# Autodesk Inventor assembly: sestava estonsko
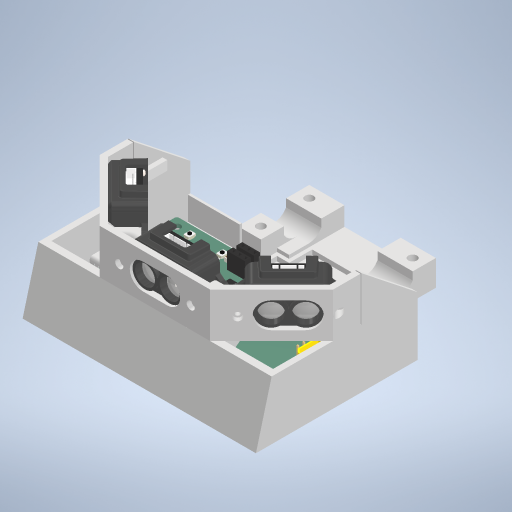
[picture p0: Inventor's stored thumbnail of the model, 512x512]
Saved by Autodesk Inventor 2024 (Build 280153000, 153)
## iProperties
Created: 2023-10-31
Part Number: sestava estonsko
Document SubType Name: Assembly
Designer: Simak
Author: Simak
## Documents named in this file (4)
- C:\Users\jaryj\Desktop\Škola\Mini sumo\RoboCop\- 3D -\wip\sestava estonsko.iam
- C:\Users\jaryj\Desktop\Škola\Mini sumo\RoboCop\- 3D -\el._parts\sumec\sumec.ipt
- C:\Users\jaryj\Desktop\Škola\Mini sumo\RoboCop\- 3D -\wip\tělo estonsko.ipt
- C:\Users\jaryj\Desktop\Škola\Mini sumo\RoboCop\- 3D -\wip\Sestava TF-Luna a držáku.iam
## Components (3 placed, 3 different names)
1. tělo estonsko:1 — Proti sobě:1, Vložit:1, Vložit:2, Tuhé:1
2. sumec:1 — Proti sobě:1, Vložit:1, Vložit:2
3. Sestava TF-Luna a držáku:1 [sub-assembly] — Tuhé:1
## Relationships (4: Insert 2, Mate 1, WeldJoint 1)
- Proti sobě:1 [Mate] (4 mm): tělo estonsko:1 ↔ sumec:1
- Vložit:1 [Insert]: tělo estonsko:1 ↔ sumec:1
- Vložit:2 [Insert]: tělo estonsko:1 ↔ sumec:1
- Tuhé:1 [WeldJoint]: tělo estonsko:1 ↔ Sestava TF-Luna a držáku:1
